# Autodesk Inventor assembly: GEM Gear Box ans Gears
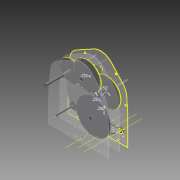
[picture p0: Inventor's stored thumbnail of the model, 180x180]
Saved by Autodesk Inventor 2012 (Build 160160000, 160)
## iProperties
Created: 2012-04-29
Part Number: GEM Gear Box ans Gears
Document SubType Name: Assembly
Designer: gdkaine
Author: gdkaine
## Documents named in this file (10)
- C:\Users\gdkaine\Documents\GEM Gear Box ans Gears.iam
- C:\Users\gdkaine\Documents\GEM Gear Mount Right.ipt
- C:\Users\gdkaine\Documents\GEM Gear Mount.ipt
- C:\Users\gdkaine\Documents\GEM Gear Mount Left.ipt
- C:\Users\gdkaine\Documents\GEM Gear Box ans Gears\Design Accelerator\Spur Gears1.iam
- C:\Users\gdkaine\Documents\GEM Gear Box ans Gears\Design Accelerator\Spur Gears2.iam
- C:\Users\gdkaine\Documents\GEM Gear Box ans Gears\Design Accelerator\Spur Gears3.iam
- C:\Users\gdkaine\Documents\GEM Gear Box ans Gears\Design Accelerator\Spur Gears4.iam
- C:\Users\gdkaine\Documents\GEM Gear Box ans Gears\Design Accelerator\Spur Gears5.iam
- C:\Users\gdkaine\Documents\Timing belt.iam
## Components (10 placed, 5 different names)
1. GEM Gear Mount Right:1 — Flush:1, Flush:2, Mate:33, Mate:41, Mate:42
2. GEM Gear Mount:1 — Flush:1, Flush:2, Flush:3, Flush:4, Mate:18, Mate:22, Mate:23, Mate:30, Mate:37, Mate:38, Mate:39, Mate:40, Mate:41
3. GEM Gear Mount Left:1 — Flush:3, Flush:4, Mate:2, Mate:5, Mate:10, Mate:34, Mate:35, Mate:36, Mate:37
4. Spur Gears:1 [sub-assembly] — Mate:36
5. Spur Gears:2 [sub-assembly] — Mate:12, Mate:13, Mate:38
6. Spur Gears:3 [sub-assembly] — Mate:14, Mate:15, Mate:35
7. Spur Gears:4 [sub-assembly] — Mate:7, Mate:9, Mate:34
8. Spur Gears:5 [sub-assembly] — Mate:40
9. Spur Gears:6 [sub-assembly] — Mate:25, Mate:26, Mate:39
10. Timing belt:1 [sub-assembly] — Mate:33, Mate:42
## Relationships (41: Mate 37, Flush 4)
- Flush:1: GEM Gear Mount Right:1 ↔ GEM Gear Mount:1
- Flush:2: GEM Gear Mount Right:1 ↔ GEM Gear Mount:1
- Flush:3: GEM Gear Mount:1 ↔ GEM Gear Mount Left:1
- Flush:4: GEM Gear Mount:1 ↔ GEM Gear Mount Left:1
- Mate:2: GEM Gear Mount Left:1
- Mate:3
- Mate:5: GEM Gear Mount Left:1
- Mate:6
- Mate:7: Spur Gears:4
- Mate:8
- Mate:9: Spur Gears:4
- Mate:10: GEM Gear Mount Left:1
- Mate:11
- Mate:12: Spur Gears:2
- Mate:13: Spur Gears:2
- Mate:14: Spur Gears:3
- Mate:15: Spur Gears:3
- Mate:18: GEM Gear Mount:1
- Mate:19
- Mate:20
- Mate:21
- Mate:22: GEM Gear Mount:1
- Mate:23: GEM Gear Mount:1
- Mate:24
- Mate:25: Spur Gears:6
- Mate:26: Spur Gears:6
- Mate:27
- Mate:28
- Mate:29
- Mate:30: GEM Gear Mount:1
- Mate:31
- Mate:33: GEM Gear Mount Right:1 ↔ Timing belt:1
- Mate:34 (12.7 mm): GEM Gear Mount Left:1 ↔ Spur Gears:4
- Mate:35 (25.4 mm): GEM Gear Mount Left:1 ↔ Spur Gears:3
- Mate:36 (38.1 mm): GEM Gear Mount Left:1 ↔ Spur Gears:1
- Mate:37 (50.8 mm): GEM Gear Mount:1 ↔ GEM Gear Mount Left:1
- Mate:38 (12.7 mm): GEM Gear Mount:1 ↔ Spur Gears:2
- Mate:39 (25.4 mm): GEM Gear Mount:1 ↔ Spur Gears:6
- Mate:40 (25.4 mm): GEM Gear Mount:1 ↔ Spur Gears:5
- Mate:41 (38.1 mm): GEM Gear Mount Right:1 ↔ GEM Gear Mount:1
- Mate:42: GEM Gear Mount Right:1 ↔ Timing belt:1
